# Autodesk Inventor assembly: Pancake_Assy
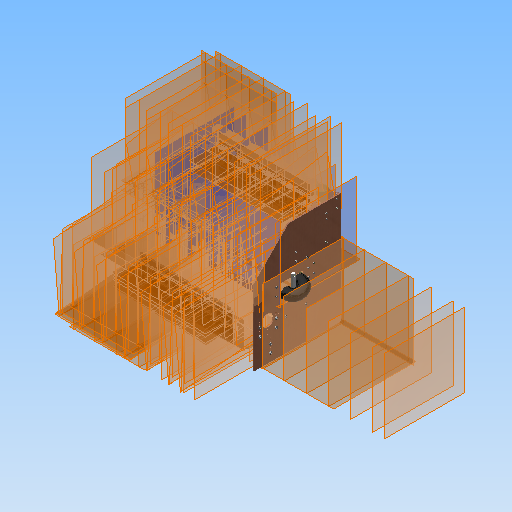
[picture p0: Inventor's stored thumbnail of the model, 512x512]
Saved by Autodesk Inventor 2018.1 (Build 221171000, 171)
## iProperties
Created: 2019-02-21
Part Number: Pancake_Assy
Document SubType Name: Assembly
Designer: James
Author: James
## Documents named in this file (19)
- C:\Users\admin\Desktop\Ball Sorting Machine\Ball-Sorting-Machine\Pancake Sort\Pancake_Assy.iam
- C:\Users\admin\Desktop\Ball Sorting Machine\Ball-Sorting-Machine\Pancake Sort\Pancake_LHS.ipt
- C:\Users\admin\Desktop\Ball Sorting Machine\Ball-Sorting-Machine\Pancake Sort\Pancake_Catch Assy.iam
- C:\Users\admin\Desktop\Ball Sorting Machine\Ball-Sorting-Machine\Pancake Sort\Nyloc Nut - M4.ipt
- C:\Users\admin\Desktop\Ball Sorting Machine\Ball-Sorting-Machine\Pancake Sort\Socket Cap Screw - Standard - (A2) - M4 x 16.ipt
- C:\Users\admin\Desktop\Ball Sorting Machine\Ball-Sorting-Machine\Pancake Sort\Pancake_Top Board Assy.iam
- C:\Users\admin\Desktop\Ball Sorting Machine\Ball-Sorting-Machine\Selection Sort\Ball 30mm.ipt
- C:\Users\admin\Desktop\Ball Sorting Machine\Ball-Sorting-Machine\Pancake Sort\Pancake_Timing Assy.iam
- C:\Users\admin\Desktop\Ball Sorting Machine\Ball-Sorting-Machine\Pancake Sort\Locknut - M3.ipt
- C:\Users\admin\Desktop\Ball Sorting Machine\Ball-Sorting-Machine\Pancake Sort\Socket Cap Screw - Standard - (A2) - M3 x 16.ipt
- C:\Users\admin\Desktop\Ball Sorting Machine\Ball-Sorting-Machine\Pancake Sort\Pancake_Drop Assy.iam
- C:\Users\admin\Desktop\Ball Sorting Machine\Ball-Sorting-Machine\Pancake Sort\Pancake_Exit Assy.iam
- C:\Users\admin\Desktop\Ball Sorting Machine\Ball-Sorting-Machine\Pancake Sort\Pancake_Tilted Tube Assy.iam
- C:\Users\admin\Desktop\Ball Sorting Machine\Ball-Sorting-Machine\Pancake Sort\Pancake_Flexi Pipe Assy.iam
- C:\Users\admin\Desktop\Ball Sorting Machine\Ball-Sorting-Machine\Pancake Sort\Pancake_Flexi Pipe Assy Flipped.iam
- C:\Users\admin\Desktop\Ball Sorting Machine\Ball-Sorting-Machine\Pancake Sort\Pancake_Tilted Tube Assy 2.iam
- C:\Users\admin\Desktop\Ball Sorting Machine\Ball-Sorting-Machine\Pancake Sort\Pancake_Timing Assy 2.iam
- C:\Users\admin\Desktop\Ball Sorting Machine\Ball-Sorting-Machine\Pancake Sort\Pancake_Reverse Assy.iam
- C:\Users\admin\Desktop\Ball Sorting Machine\Ball-Sorting-Machine\Pancake Sort\Pancake_Floor Bracket.ipt
## Components (70 placed, 18 different names)
1. Pancake_LHS:1 — Flush:1, Flush:2, Flush:3, Mate:3, Mate:5, Mate:6, Mate:8, Mate:9, Mate:10, Mate:11, Mate:24, Mate:26, Mate:27, Mate:30, Mate:31, Mate:32, Mate:33, Mate:34, Mate:35, Mate:36, Mate:39, Mate:40, Mate:51, Mate:52, Mate:53, Mate:54, Mate:75, Mate:76, Mate:83, Mate:84, Mate:90, Mate:91, Mate:92, Mate:93, Mate:102, Mate:103, Mate:148, Mate:149, Mate:150, Mate:151, Mate:153, Mate:154, Mate:155, Mate:156, Mate:157, Mate:160, Mate:161, Mate:164, Mate:165, Mate:166, Mate:167, Mate:168, Mate:169, Mate:170, Mate:158, Mate:159
2. Pancake_LHS:2 — Flush:4, Flush:5, Mate:4, Mate:7, Mate:16, Mate:17, Mate:18, Mate:19, Mate:25, Mate:28, Mate:29, Mate:43, Mate:44, Mate:47, Mate:48, Mate:59, Mate:60, Mate:63, Mate:64, Mate:81, Mate:82, Mate:85, Mate:98, Mate:99, Mate:106, Mate:137, Mate:138, Mate:139, Mate:140, Mate:141, Mate:142, Mate:143, Mate:144, Mate:145, Mate:146, Mate:147, Mate:152
3. Pancake_Catch Assy:1 [sub-assembly] — Mate:3, Mate:4, Mate:5, Mate:6, Mate:7, Mate:12, Mate:13, Mate:20, Mate:21
4. Pancake_Top Board Assy:1 [sub-assembly] — Mate:24, Mate:25, Mate:26, Mate:27, Mate:28, Tangent:1, Tangent:2, Mate:71, Mate:72, Mate:73, Mate:74, Mate:77, Mate:78, Mate:79, Mate:80
5. Ball 30mm:1 — Tangent:1
6. Ball 30mm:2 — Tangent:2
7. Pancake_Timing Assy:1 [sub-assembly] — Flush:6, Mate:29, Mate:30, Mate:31, Mate:32, Mate:33, Mate:34, Mate:37, Mate:41, Mate:45, Mate:46, Mate:55, Mate:56, Mate:61, Mate:62
8. Pancake_Drop Assy:1 [sub-assembly] — Flush:7, Mate:83, Mate:84, Mate:85, Mate:94, Mate:95, Mate:96, Mate:97, Mate:100, Mate:101
9. Pancake_Exit Assy:1 [sub-assembly] — Flush:8, Mate:102, Mate:103, Mate:106, Mate:115, Mate:116, Mate:121, Mate:122, Mate:123, Mate:124, Mate:127, Mate:128, Mate:131, Mate:132, Tangent:5
10. Pancake_Tilted Tube Assy:1 [sub-assembly] — Mate:139, Mate:140, Mate:141
11. Pancake_Tilted Tube Assy 2:1 [sub-assembly] — Mate:142, Mate:146, Mate:147, Tangent:4
12. Pancake_Flexi Pipe Assy:1 [sub-assembly] — Mate:143, Mate:144, Mate:145
13. Pancake_Flexi Pipe Assy Flipped:1 [sub-assembly] — Mate:148, Mate:149, Mate:150
14. Ball 30mm:4 — Tangent:4
15. Pancake_Timing Assy 2:1 [sub-assembly] — Mate:151, Mate:152, Mate:160, Mate:161
16. Pancake_Reverse Assy:1 [sub-assembly] — Mate:153, Mate:154, Mate:155, Mate:156, Mate:157, Mate:158, Mate:159
17. Ball 30mm:5 — Tangent:5
18. Pancake_Floor Bracket:1 — Mate:164, Mate:165, Mate:166, Mate:171, Mate:172
19. Nyloc Nut - M4:23 — Mate:171, Mate:174
20. Socket Cap Screw - Standard - (A2) - M4 x 16:23 — Mate:167, Mate:169, Mate:174
21. Nyloc Nut - M4:24 — Mate:172, Mate:173
22. Socket Cap Screw - Standard - (A2) - M4 x 16:24 — Mate:168, Mate:170, Mate:173
23. Nyloc Nut - M4:17 — Mate:123
24. Socket Cap Screw - Standard - (A2) - M4 x 16:17 — Mate:115, Mate:122
25. Nyloc Nut - M4:18 — Mate:124
26. Socket Cap Screw - Standard - (A2) - M4 x 16:18 — Mate:116, Mate:121
27. Nyloc Nut - M4:21 — Mate:138
28. Socket Cap Screw - Standard - (A2) - M4 x 16:21 — Mate:127, Mate:131
29. Nyloc Nut - M4:22 — Mate:137
30. Socket Cap Screw - Standard - (A2) - M4 x 16:22 — Mate:128, Mate:132
31. Nyloc Nut - M4:13 — Mate:94
32. Socket Cap Screw - Standard - (A2) - M4 x 16:13 — Mate:90, Mate:93
33. Nyloc Nut - M4:14 — Mate:95
34. Socket Cap Screw - Standard - (A2) - M4 x 16:14 — Mate:91, Mate:92
35. Nyloc Nut - M4:15 — Mate:101
36. Socket Cap Screw - Standard - (A2) - M4 x 16:15 — Mate:97, Mate:99
37. Nyloc Nut - M4:16 — Mate:100
38. Socket Cap Screw - Standard - (A2) - M4 x 16:16 — Mate:96, Mate:98
39. Nyloc Nut - M4:5 — Mate:37, Mate:38
40. Socket Cap Screw - Standard - (A2) - M4 x 16:5 — Mate:35, Mate:36, Mate:38
41. Nyloc Nut - M4:6 — Mate:41, Mate:42
42. Socket Cap Screw - Standard - (A2) - M4 x 16:6 — Mate:39, Mate:40, Mate:42
43. Nyloc Nut - M4:7 — Mate:46, Mate:50
44. Socket Cap Screw - Standard - (A2) - M4 x 16:7 — Mate:43, Mate:47, Mate:49
45. Nyloc Nut - M4:8 — Mate:45, Mate:49
46. Socket Cap Screw - Standard - (A2) - M4 x 16:8 — Mate:44, Mate:48, Mate:50
47. Locknut - M3:1 — Mate:53, Mate:57
48. Socket Cap Screw - Standard - (A2) - M3 x 16:1 — Mate:51, Mate:55, Mate:57
49. Locknut - M3:2 — Mate:54, Mate:58
50. Socket Cap Screw - Standard - (A2) - M3 x 16:2 — Mate:52, Mate:56, Mate:58
51. Locknut - M3:3 — Mate:63, Mate:65
52. Socket Cap Screw - Standard - (A2) - M3 x 16:3 — Mate:59, Mate:61, Mate:66
53. Locknut - M3:4 — Mate:64, Mate:66
54. Socket Cap Screw - Standard - (A2) - M3 x 16:4 — Mate:60, Mate:62, Mate:65
55. Nyloc Nut - M4:9 — Mate:76
56. Socket Cap Screw - Standard - (A2) - M4 x 16:9 — Mate:71, Mate:73
57. Nyloc Nut - M4:10 — Mate:75
58. Socket Cap Screw - Standard - (A2) - M4 x 16:10 — Mate:72, Mate:74
59. Nyloc Nut - M4:11 — Mate:77, Mate:81
60. Socket Cap Screw - Standard - (A2) - M4 x 16:11 — Mate:79
61. Nyloc Nut - M4:12 — Mate:82
62. Socket Cap Screw - Standard - (A2) - M4 x 16:12 — Mate:78, Mate:80
63. Nyloc Nut - M4:1 — Mate:20, Mate:23
64. Socket Cap Screw - Standard - (A2) - M4 x 16:1 — Mate:16, Mate:19, Mate:22
65. Nyloc Nut - M4:2 — Mate:21, Mate:22
66. Socket Cap Screw - Standard - (A2) - M4 x 16:2 — Mate:17, Mate:18, Mate:23
67. Nyloc Nut - M4:3 — Mate:12, Mate:15
68. Socket Cap Screw - Standard - (A2) - M4 x 16:3 — Mate:8, Mate:11, Mate:15
69. Nyloc Nut - M4:4 — Mate:13, Mate:14
70. Socket Cap Screw - Standard - (A2) - M4 x 16:4 — Mate:9, Mate:10, Mate:14
## Relationships (164: Mate 152, Flush 8, Tangent 4)
- Flush:1: Pancake_LHS:1
- Flush:2: Pancake_LHS:1
- Flush:3: Pancake_LHS:1
- Flush:4: Pancake_LHS:2
- Flush:5: Pancake_LHS:2
- Mate:3: Pancake_LHS:1 ↔ Pancake_Catch Assy:1
- Mate:4: Pancake_LHS:2 ↔ Pancake_Catch Assy:1
- Mate:5: Pancake_LHS:1 ↔ Pancake_Catch Assy:1
- Mate:6: Pancake_LHS:1 ↔ Pancake_Catch Assy:1
- Mate:7: Pancake_LHS:2 ↔ Pancake_Catch Assy:1
- Mate:8: Pancake_LHS:1 ↔ Socket Cap Screw - Standard - (A2) - M4 x 16:3
- Mate:9: Pancake_LHS:1 ↔ Socket Cap Screw - Standard - (A2) - M4 x 16:4
- Mate:10: Pancake_LHS:1 ↔ Socket Cap Screw - Standard - (A2) - M4 x 16:4
- Mate:11: Pancake_LHS:1 ↔ Socket Cap Screw - Standard - (A2) - M4 x 16:3
- Mate:12: Pancake_Catch Assy:1 ↔ Nyloc Nut - M4:3
- Mate:13: Pancake_Catch Assy:1 ↔ Nyloc Nut - M4:4
- Mate:14: Nyloc Nut - M4:4 ↔ Socket Cap Screw - Standard - (A2) - M4 x 16:4
- Mate:15: Nyloc Nut - M4:3 ↔ Socket Cap Screw - Standard - (A2) - M4 x 16:3
- Mate:16: Pancake_LHS:2 ↔ Socket Cap Screw - Standard - (A2) - M4 x 16:1
- Mate:17: Pancake_LHS:2 ↔ Socket Cap Screw - Standard - (A2) - M4 x 16:2
- Mate:18: Pancake_LHS:2 ↔ Socket Cap Screw - Standard - (A2) - M4 x 16:2
- Mate:19: Pancake_LHS:2 ↔ Socket Cap Screw - Standard - (A2) - M4 x 16:1
- Mate:20: Pancake_Catch Assy:1 ↔ Nyloc Nut - M4:1
- Mate:21: Pancake_Catch Assy:1 ↔ Nyloc Nut - M4:2
- Mate:22: Socket Cap Screw - Standard - (A2) - M4 x 16:1 ↔ Nyloc Nut - M4:2
- Mate:23: Nyloc Nut - M4:1 ↔ Socket Cap Screw - Standard - (A2) - M4 x 16:2
- Mate:24: Pancake_LHS:1 ↔ Pancake_Top Board Assy:1
- Mate:25: Pancake_LHS:2 ↔ Pancake_Top Board Assy:1
- Mate:26: Pancake_LHS:1 ↔ Pancake_Top Board Assy:1
- Mate:27: Pancake_LHS:1 ↔ Pancake_Top Board Assy:1
- Mate:28: Pancake_LHS:2 ↔ Pancake_Top Board Assy:1
- Tangent:1: Pancake_Top Board Assy:1 ↔ Ball 30mm:1
- Tangent:2: Pancake_Top Board Assy:1 ↔ Ball 30mm:2
- Flush:6: Pancake_Timing Assy:1
- Mate:29: Pancake_LHS:2 ↔ Pancake_Timing Assy:1
- Mate:30: Pancake_LHS:1 ↔ Pancake_Timing Assy:1
- Mate:31: Pancake_LHS:1 ↔ Pancake_Timing Assy:1
- Mate:32: Pancake_LHS:1 ↔ Pancake_Timing Assy:1
- Mate:33: Pancake_LHS:1 ↔ Pancake_Timing Assy:1
- Mate:34: Pancake_LHS:1 ↔ Pancake_Timing Assy:1
- Mate:35: Pancake_LHS:1 ↔ Socket Cap Screw - Standard - (A2) - M4 x 16:5
- Mate:36: Pancake_LHS:1 ↔ Socket Cap Screw - Standard - (A2) - M4 x 16:5
- Mate:37: Pancake_Timing Assy:1 ↔ Nyloc Nut - M4:5
- Mate:38: Nyloc Nut - M4:5 ↔ Socket Cap Screw - Standard - (A2) - M4 x 16:5
- Mate:39: Pancake_LHS:1 ↔ Socket Cap Screw - Standard - (A2) - M4 x 16:6
- Mate:40: Pancake_LHS:1 ↔ Socket Cap Screw - Standard - (A2) - M4 x 16:6
- Mate:41: Pancake_Timing Assy:1 ↔ Nyloc Nut - M4:6
- Mate:42: Nyloc Nut - M4:6 ↔ Socket Cap Screw - Standard - (A2) - M4 x 16:6
- Mate:43: Pancake_LHS:2 ↔ Socket Cap Screw - Standard - (A2) - M4 x 16:7
- Mate:44: Pancake_LHS:2 ↔ Socket Cap Screw - Standard - (A2) - M4 x 16:8
- Mate:45: Pancake_Timing Assy:1 ↔ Nyloc Nut - M4:8
- Mate:46: Pancake_Timing Assy:1 ↔ Nyloc Nut - M4:7
- Mate:47: Pancake_LHS:2 ↔ Socket Cap Screw - Standard - (A2) - M4 x 16:7
- Mate:48: Pancake_LHS:2 ↔ Socket Cap Screw - Standard - (A2) - M4 x 16:8
- Mate:49: Socket Cap Screw - Standard - (A2) - M4 x 16:7 ↔ Nyloc Nut - M4:8
- Mate:50: Nyloc Nut - M4:7 ↔ Socket Cap Screw - Standard - (A2) - M4 x 16:8
- Mate:51: Pancake_LHS:1 ↔ Socket Cap Screw - Standard - (A2) - M3 x 16:1
- Mate:52: Pancake_LHS:1 ↔ Socket Cap Screw - Standard - (A2) - M3 x 16:2
- Mate:53: Pancake_LHS:1 ↔ Locknut - M3:1
- Mate:54: Pancake_LHS:1 ↔ Locknut - M3:2
- Mate:55: Pancake_Timing Assy:1 ↔ Socket Cap Screw - Standard - (A2) - M3 x 16:1
- Mate:56: Pancake_Timing Assy:1 ↔ Socket Cap Screw - Standard - (A2) - M3 x 16:2
- Mate:57: Locknut - M3:1 ↔ Socket Cap Screw - Standard - (A2) - M3 x 16:1
- Mate:58: Locknut - M3:2 ↔ Socket Cap Screw - Standard - (A2) - M3 x 16:2
- Mate:59: Pancake_LHS:2 ↔ Socket Cap Screw - Standard - (A2) - M3 x 16:3
- Mate:60: Pancake_LHS:2 ↔ Socket Cap Screw - Standard - (A2) - M3 x 16:4
- Mate:61: Pancake_Timing Assy:1 ↔ Socket Cap Screw - Standard - (A2) - M3 x 16:3
- Mate:62: Pancake_Timing Assy:1 ↔ Socket Cap Screw - Standard - (A2) - M3 x 16:4
- Mate:63: Pancake_LHS:2 ↔ Locknut - M3:3
- Mate:64: Pancake_LHS:2 ↔ Locknut - M3:4
- Mate:65: Locknut - M3:3 ↔ Socket Cap Screw - Standard - (A2) - M3 x 16:4
- Mate:66: Socket Cap Screw - Standard - (A2) - M3 x 16:3 ↔ Locknut - M3:4
- [Mate]: Nyloc Nut - M4:9 ↔ Socket Cap Screw - Standard - (A2) - M4 x 16:9
- [Mate]: Nyloc Nut - M4:10 ↔ Socket Cap Screw - Standard - (A2) - M4 x 16:10
- [Mate]: Nyloc Nut - M4:11 ↔ Socket Cap Screw - Standard - (A2) - M4 x 16:11
- [Mate]: Nyloc Nut - M4:12 ↔ Socket Cap Screw - Standard - (A2) - M4 x 16:12
- Mate:71: Pancake_Top Board Assy:1 ↔ Socket Cap Screw - Standard - (A2) - M4 x 16:9
- Mate:72: Pancake_Top Board Assy:1 ↔ Socket Cap Screw - Standard - (A2) - M4 x 16:10
- Mate:73: Pancake_Top Board Assy:1 ↔ Socket Cap Screw - Standard - (A2) - M4 x 16:9
- Mate:74: Pancake_Top Board Assy:1 ↔ Socket Cap Screw - Standard - (A2) - M4 x 16:10
- Mate:75: Pancake_LHS:1 ↔ Nyloc Nut - M4:10
- Mate:76: Pancake_LHS:1 ↔ Nyloc Nut - M4:9
- Mate:77: Pancake_Top Board Assy:1 ↔ Nyloc Nut - M4:11
- Mate:78: Pancake_Top Board Assy:1 ↔ Socket Cap Screw - Standard - (A2) - M4 x 16:12
- Mate:79: Pancake_Top Board Assy:1 ↔ Socket Cap Screw - Standard - (A2) - M4 x 16:11
- Mate:80: Pancake_Top Board Assy:1 ↔ Socket Cap Screw - Standard - (A2) - M4 x 16:12
- Mate:81: Pancake_LHS:2 ↔ Nyloc Nut - M4:11
- Mate:82: Pancake_LHS:2 ↔ Nyloc Nut - M4:12
- Flush:7: Pancake_Drop Assy:1
- Mate:83: Pancake_LHS:1 ↔ Pancake_Drop Assy:1
- Mate:84: Pancake_LHS:1 ↔ Pancake_Drop Assy:1
- Mate:85: Pancake_LHS:2 ↔ Pancake_Drop Assy:1
- [Mate]: Nyloc Nut - M4:13 ↔ Socket Cap Screw - Standard - (A2) - M4 x 16:13
- [Mate]: Nyloc Nut - M4:14 ↔ Socket Cap Screw - Standard - (A2) - M4 x 16:14
- [Mate]: Nyloc Nut - M4:15 ↔ Socket Cap Screw - Standard - (A2) - M4 x 16:15
- [Mate]: Nyloc Nut - M4:16 ↔ Socket Cap Screw - Standard - (A2) - M4 x 16:16
- Mate:90: Pancake_LHS:1 ↔ Socket Cap Screw - Standard - (A2) - M4 x 16:13
- Mate:91: Pancake_LHS:1 ↔ Socket Cap Screw - Standard - (A2) - M4 x 16:14
- Mate:92: Pancake_LHS:1 ↔ Socket Cap Screw - Standard - (A2) - M4 x 16:14
- Mate:93: Pancake_LHS:1 ↔ Socket Cap Screw - Standard - (A2) - M4 x 16:13
- Mate:94: Pancake_Drop Assy:1 ↔ Nyloc Nut - M4:13
- Mate:95: Pancake_Drop Assy:1 ↔ Nyloc Nut - M4:14
- Mate:96: Pancake_Drop Assy:1 ↔ Socket Cap Screw - Standard - (A2) - M4 x 16:16
- Mate:97: Pancake_Drop Assy:1 ↔ Socket Cap Screw - Standard - (A2) - M4 x 16:15
- Mate:98: Pancake_LHS:2 ↔ Socket Cap Screw - Standard - (A2) - M4 x 16:16
- Mate:99: Pancake_LHS:2 ↔ Socket Cap Screw - Standard - (A2) - M4 x 16:15
- Mate:100: Pancake_Drop Assy:1 ↔ Nyloc Nut - M4:16
- Mate:101: Pancake_Drop Assy:1 ↔ Nyloc Nut - M4:15
- Flush:8: Pancake_Exit Assy:1
- Mate:102: Pancake_LHS:1 ↔ Pancake_Exit Assy:1
- Mate:103: Pancake_LHS:1 ↔ Pancake_Exit Assy:1
- Mate:106: Pancake_LHS:2 ↔ Pancake_Exit Assy:1
- [Mate]: Nyloc Nut - M4:17 ↔ Socket Cap Screw - Standard - (A2) - M4 x 16:17
- [Mate]: Nyloc Nut - M4:18 ↔ Socket Cap Screw - Standard - (A2) - M4 x 16:18
- [Mate]: Nyloc Nut - M4:21 ↔ Socket Cap Screw - Standard - (A2) - M4 x 16:21
- [Mate]: Nyloc Nut - M4:22 ↔ Socket Cap Screw - Standard - (A2) - M4 x 16:22
- Mate:115: Pancake_Exit Assy:1 ↔ Socket Cap Screw - Standard - (A2) - M4 x 16:17
- Mate:116: Pancake_Exit Assy:1 ↔ Socket Cap Screw - Standard - (A2) - M4 x 16:18
- Mate:121: Pancake_Exit Assy:1 ↔ Socket Cap Screw - Standard - (A2) - M4 x 16:18
- Mate:122: Pancake_Exit Assy:1 ↔ Socket Cap Screw - Standard - (A2) - M4 x 16:17
- Mate:123 (5 mm): Pancake_Exit Assy:1 ↔ Nyloc Nut - M4:17
- Mate:124 (5 mm): Pancake_Exit Assy:1 ↔ Nyloc Nut - M4:18
- Mate:127: Pancake_Exit Assy:1 ↔ Socket Cap Screw - Standard - (A2) - M4 x 16:21
- Mate:128: Pancake_Exit Assy:1 ↔ Socket Cap Screw - Standard - (A2) - M4 x 16:22
- Mate:131: Pancake_Exit Assy:1 ↔ Socket Cap Screw - Standard - (A2) - M4 x 16:21
- Mate:132: Pancake_Exit Assy:1 ↔ Socket Cap Screw - Standard - (A2) - M4 x 16:22
- Mate:137: Pancake_LHS:2 ↔ Nyloc Nut - M4:22
- Mate:138: Pancake_LHS:2 ↔ Nyloc Nut - M4:21
- Mate:139: Pancake_LHS:2 ↔ Pancake_Tilted Tube Assy:1
- Mate:140: Pancake_LHS:2 ↔ Pancake_Tilted Tube Assy:1
- Mate:141: Pancake_LHS:2 ↔ Pancake_Tilted Tube Assy:1
- Mate:142: Pancake_LHS:2 ↔ Pancake_Tilted Tube Assy 2:1
- Mate:143: Pancake_LHS:2 ↔ Pancake_Flexi Pipe Assy:1
- Mate:144: Pancake_LHS:2 ↔ Pancake_Flexi Pipe Assy:1
- Mate:145: Pancake_LHS:2 ↔ Pancake_Flexi Pipe Assy:1
- Mate:146: Pancake_LHS:2 ↔ Pancake_Tilted Tube Assy 2:1
- Mate:147: Pancake_LHS:2 ↔ Pancake_Tilted Tube Assy 2:1
- Mate:148: Pancake_LHS:1 ↔ Pancake_Flexi Pipe Assy Flipped:1
- Mate:149: Pancake_LHS:1 ↔ Pancake_Flexi Pipe Assy Flipped:1
- Mate:150: Pancake_LHS:1 ↔ Pancake_Flexi Pipe Assy Flipped:1
- Tangent:4: Pancake_Tilted Tube Assy 2:1 ↔ Ball 30mm:4
- Mate:151: Pancake_LHS:1 ↔ Pancake_Timing Assy 2:1
- Mate:152: Pancake_LHS:2 ↔ Pancake_Timing Assy 2:1
- Mate:153: Pancake_LHS:1 ↔ Pancake_Reverse Assy:1
- Mate:154: Pancake_LHS:1 ↔ Pancake_Reverse Assy:1
- Mate:155: Pancake_LHS:1 ↔ Pancake_Reverse Assy:1
- Mate:156: Pancake_LHS:1 ↔ Pancake_Reverse Assy:1
- Mate:157: Pancake_LHS:1 ↔ Pancake_Reverse Assy:1
- Mate:158: Pancake_LHS:1 ↔ Pancake_Reverse Assy:1
- Mate:159: Pancake_LHS:1 ↔ Pancake_Reverse Assy:1
- Mate:160: Pancake_LHS:1 ↔ Pancake_Timing Assy 2:1
- Mate:161: Pancake_LHS:1 ↔ Pancake_Timing Assy 2:1
- Tangent:5: Pancake_Exit Assy:1 ↔ Ball 30mm:5
- Mate:164: Pancake_LHS:1 ↔ Pancake_Floor Bracket:1
- Mate:165: Pancake_LHS:1 ↔ Pancake_Floor Bracket:1
- Mate:166: Pancake_LHS:1 ↔ Pancake_Floor Bracket:1
- Mate:167: Pancake_LHS:1 ↔ Socket Cap Screw - Standard - (A2) - M4 x 16:23
- Mate:168: Pancake_LHS:1 ↔ Socket Cap Screw - Standard - (A2) - M4 x 16:24
- Mate:169: Pancake_LHS:1 ↔ Socket Cap Screw - Standard - (A2) - M4 x 16:23
- Mate:170: Pancake_LHS:1 ↔ Socket Cap Screw - Standard - (A2) - M4 x 16:24
- Mate:171: Pancake_Floor Bracket:1 ↔ Nyloc Nut - M4:23
- Mate:172: Pancake_Floor Bracket:1 ↔ Nyloc Nut - M4:24
- Mate:173: Nyloc Nut - M4:24 ↔ Socket Cap Screw - Standard - (A2) - M4 x 16:24
- Mate:174: Nyloc Nut - M4:23 ↔ Socket Cap Screw - Standard - (A2) - M4 x 16:23
## Named parameters: d75_d46 = 0 mm, d76_d46 = 0 mm, d77_d46 = 0 mm, d78_d46 = 0 mm, d97_d75_d46 = 0 mm, d98_d75_d46 = 0 mm, d99_d75_d46 = 0 mm, d100_d75_d46 = 0 mm, d120_d76_d46 = 0 mm, d121_d76_d46 = 0 mm, d124_d76_d46 = 0 mm, d125_d76_d46 = 0 mm
